# Autodesk Inventor assembly: Brain_for_kickstarter_video_demo
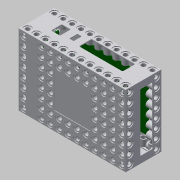
[picture p0: Inventor's stored thumbnail of the model, 180x180]
Saved by Autodesk Inventor 2019.3 (Build 233278000, 278)
## iProperties
Created: 2019-04-11
Part Number: Brain_for_kickstarter_video_demo
Document SubType Name: Assembly
Designer: Varga Daniel
Author: Varga Daniel
## Documents named in this file (9)
- C:\!_Dani\!_cloud\OneDrive\!_munka\Revolution\RevvyDemoKit\Structural parts\Kickstarter videos\Brain pcb\Brain_for_kickstarter_video_demo.iam
- C:\!_Dani\!_cloud\OneDrive\!_munka\Revolution\RevvyDemoKit\Structural parts\Kickstarter videos\Brain pcb\BRcA_1.ipt
- C:\!_Dani\!_cloud\OneDrive\!_munka\Revolution\RevvyDemoKit\Structural parts\Kickstarter videos\Brain pcb\BRcA_3.ipt
- C:\!_Dani\!_cloud\OneDrive\!_munka\Revolution\RevvyDemoKit\Structural parts\Kickstarter videos\Brain pcb\Transparent_window.ipt
- C:\!_Dani\!_cloud\OneDrive\!_munka\Revolution\RevvyDemoKit\Structural parts\Kickstarter videos\Brain pcb\JHY_813270_2000mAh.ipt
- C:\!_Dani\!_cloud\OneDrive\!_munka\Revolution\RevvyDemoKit\Structural parts\Kickstarter videos\Brain pcb\BRcA_2_with_microphone_plug.ipt
- c:\!_Dani\!_cloud\OneDrive\!_munka\Revolution\RevvyDemoKit\Structural parts\Kickstarter videos\Brain pcb\Brain_demo_PCB.ipt
- c:\!_Dani\!_cloud\OneDrive\!_munka\Revolution\RevvyDemoKit\Structural parts\Kickstarter videos\Brain pcb\LCD_panel_demo.ipt
- c:\!_Dani\!_cloud\OneDrive\!_munka\Revolution\RevvyDemoKit\Structural parts\Kickstarter videos\Brain pcb\Raspberry_Pi_Demo.ipt
## Components (8 placed, 8 different names)
1. BRcA_1:1 — Flush:1, Flush:2, Mate:1, Mate:16, Flush:11, Flush:12, Flush:13, Mate:17, Flush:15
2. BRcA_3:1
3. Transparent_window:1
4. JHY_813270_2000mAh:1
5. BRcA_2_with_microphone_plug:1 — Mate:16, Flush:11, Flush:12, Flush:14
6. Brain_demo_PCB:1 — Flush:13, Mate:17
7. LCD_panel_demo:1 — Flush:14
8. Raspberry_Pi_Demo:1 — Flush:15
## Relationships (10: Flush 7, Mate 3)
- Flush:1: BRcA_1:1
- Flush:2: BRcA_1:1
- Mate:1: BRcA_1:1
- Mate:16: BRcA_1:1 ↔ BRcA_2_with_microphone_plug:1
- Flush:11: BRcA_1:1 ↔ BRcA_2_with_microphone_plug:1
- Flush:12: BRcA_1:1 ↔ BRcA_2_with_microphone_plug:1
- Flush:13: BRcA_1:1 ↔ Brain_demo_PCB:1
- Mate:17: BRcA_1:1 ↔ Brain_demo_PCB:1
- Flush:14: BRcA_2_with_microphone_plug:1 ↔ LCD_panel_demo:1
- Flush:15: BRcA_1:1 ↔ Raspberry_Pi_Demo:1
